# Autodesk Inventor assembly: MiniSB ADXL Mount - Generic
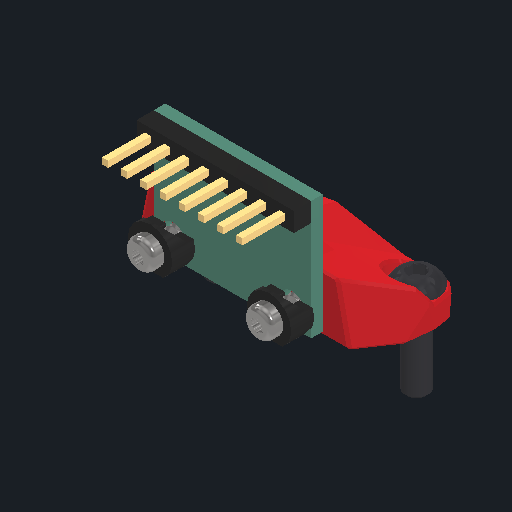
[picture p0: Inventor's stored thumbnail of the model, 512x512]
Saved by Autodesk Inventor 2025.1 (Build 291241020, 241B)
## iProperties
Created: 2025-05-09
Part Number: MiniSB ADXL Mount - Generic
Document SubType Name: Assembly
Designer: AdminForWorker
Title: MiniSB ADXL Mount - Generic
Author: AdminForWorker
## Documents named in this file (5)
- C:\Users\Joshua Eah\Documents\Voron 0.2\CAD\Master Assembly\MiniSB ADXL Mount - Generic.iam
- C:\Users\Joshua Eah\Documents\Voron 0.2\CAD\Master Assembly\ADXL345 - Generic.ipt
- C:\Users\Joshua Eah\Documents\Voron 0.2\CAD\Master Assembly\Printed Parts (25).iam
- C:\Users\Joshua Eah\Documents\Voron 0.2\CAD\Master Assembly\Hardware\M3x12 BHCS.ipt
- C:\Users\Joshua Eah\Documents\Voron 0.2\CAD\Master Assembly\Hardware\M2x10 Self Tapper.ipt
## Components (6 placed, 4 different names)
1. ADXL345 - Generic:1
2. Printed Parts (25):1 [sub-assembly] — Insert:1, Insert:2
3. M3x12 BHCS:1 — Insert:2
4. M3x12 BHCS:2 — Insert:1
5. M2x10 Self Tapper:1
6. M2x10 Self Tapper:2
## Relationships (2: Insert 2)
- Insert:1: Printed Parts (25):1 ↔ M3x12 BHCS:2
- Insert:2: Printed Parts (25):1 ↔ M3x12 BHCS:1
